# Autodesk Inventor assembly: bump thing
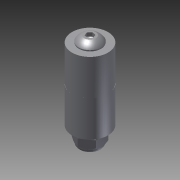
[picture p0: Inventor's stored thumbnail of the model, 180x180]
Saved by Autodesk Inventor 2014 SP1 (Build 180222100, 222)
## iProperties
Created: 2014-04-06
Part Number: bump thing
Document SubType Name: Assembly
Designer: Ryan
Author: Ryan
## Documents named in this file (4)
- C:\Users\Ryan\Desktop\sw\toss up 5th A bot\drive\bump thing.iam
- C:\Users\Ryan\Desktop\sw\lib\Aperture VEX CAD Library\Spacers\SPACER-0500-0500.ipt
- C:\Users\Ryan\Desktop\sw\lib\Aperture VEX CAD Library\Hardware\8-32\8-32 nylock.ipt
- C:\Users\Ryan\Desktop\sw\lib\Aperture VEX CAD Library\Hardware\8-32\8-23_.750.ipt
## Components (4 placed, 3 different names)
1. SPACER-0500-0500:1 — Mate:1, Mate:2, Mate:3, Mate:4, Mate:5
2. 8-32 nylock:1 — Mate:3, Mate:6
3. 8-23_.750:1 — Mate:1, Mate:2
4. SPACER-0500-0500:2 — Mate:4, Mate:5, Mate:6
## Relationships (6: Mate 6)
- Mate:1: SPACER-0500-0500:1 ↔ 8-23_.750:1
- Mate:2: SPACER-0500-0500:1 ↔ 8-23_.750:1
- Mate:3: SPACER-0500-0500:1 ↔ 8-32 nylock:1
- Mate:4: SPACER-0500-0500:1 ↔ SPACER-0500-0500:2
- Mate:5: SPACER-0500-0500:1 ↔ SPACER-0500-0500:2
- Mate:6 (1.1684 mm): 8-32 nylock:1 ↔ SPACER-0500-0500:2
